# Autodesk Inventor assembly: Assembly
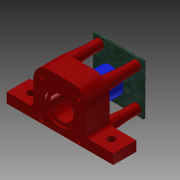
[picture p0: Inventor's stored thumbnail of the model, 180x180]
Saved by Autodesk Inventor 2014 (Build 180170000, 170)
## iProperties
Created: 2014-02-09
Part Number: Assembly
Document SubType Name: Assembly
Designer: Spooner
Author: Spooner
## Documents named in this file (5)
- C:\Users\Spooner\Documents\Inventor\ams AS514B Rotary Encoder Igus Mount\Assembly.iam
- C:\Users\Spooner\Documents\Inventor\ams AS514B Rotary Encoder Igus Mount\Igus Bracket.ipt
- C:\Users\Spooner\Documents\Inventor\ams AS514B Rotary Encoder Igus Mount\Board.ipt
- C:\Users\Spooner\Documents\Inventor\ams AS514B Rotary Encoder Igus Mount\Magnet to Igus adapter.ipt
- C:\Users\Spooner\Documents\Inventor\ams AS514B Rotary Encoder Igus Mount\Magnet.ipt
## Components (4 placed, 4 different names)
1. Igus Bracket:1 — Insert:5, Insert:6
2. Magnet to Igus adapter:1 — Insert:4
3. Magnet:1 — Insert:4, Mate:1
4. Board:1 — Mate:1, Insert:5, Insert:6
## Relationships (4: Insert 3, Mate 1)
- Insert:4: Magnet to Igus adapter:1 ↔ Magnet:1
- Mate:1 (1 mm): Magnet:1 ↔ Board:1
- Insert:5: Igus Bracket:1 ↔ Board:1
- Insert:6: Igus Bracket:1 ↔ Board:1
